# Autodesk Inventor assembly: Joint Housing top_final
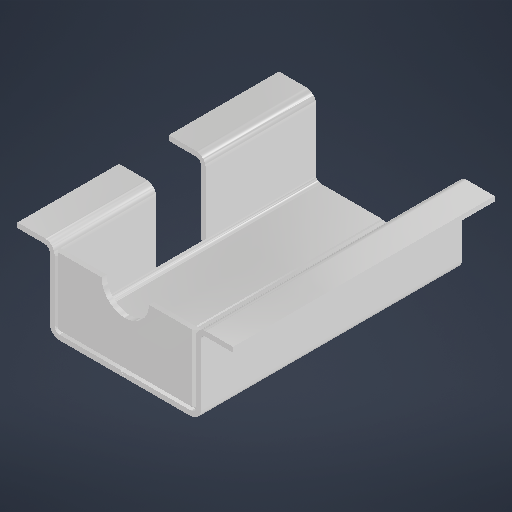
[picture p0: Inventor's stored thumbnail of the model, 512x512]
Saved by Autodesk Inventor 2026.3 (Build 303398000, 398)
## iProperties
Created: 2026-08-05
Part Number: Joint Housing top_final
Document SubType Name: Weldment
Designer: matot
Weld Material: Welded Aluminum-6061
Author: matot
## Documents named in this file (4)
- C:\Users\matot\OneDrive - Stellenbosch University\2026\MechatronicsProject478\Building the joint\Joint Assembly\Joint Housing top_final.iam
- C:\Users\matot\OneDrive - Stellenbosch University\2026\MechatronicsProject478\Building the joint\Joint Assembly\Bottom joint housing R.ipt
- C:\Users\matot\OneDrive - Stellenbosch University\2026\MechatronicsProject478\Building the joint\Joint Assembly\Bottom joint housing cover_ final.ipt
- C:\Users\matot\OneDrive - Stellenbosch University\2026\MechatronicsProject478\Building the joint\Joint Assembly\Bottom joint housing 2R.ipt
## Components (3 placed, 3 different names)
1. Bottom joint housing R:2 — Flush:3, Mate:2, Flush:4, Flush:5
2. Bottom joint housing cover_ final:1 — Flush:3, Mate:2, Mate:3
3. Bottom joint housing 2R:1 — Flush:4, Flush:5, Mate:3
## Relationships (5: Flush 3, Mate 2)
- Flush:3: Bottom joint housing R:2 ↔ Bottom joint housing cover_ final:1
- Mate:2: Bottom joint housing R:2 ↔ Bottom joint housing cover_ final:1
- Flush:4: Bottom joint housing R:2 ↔ Bottom joint housing 2R:1
- Flush:5: Bottom joint housing R:2 ↔ Bottom joint housing 2R:1
- Mate:3: Bottom joint housing cover_ final:1 ↔ Bottom joint housing 2R:1
